# Autodesk Inventor assembly: CNC-FullAssembly
(part 2 of 2)
- Mate:203: SFU1605-BallScrew500mm:2 ↔ BF12-BallScrewStabilizer2:2
- Mate:204: SFU1605-BallScrew500mm:2 ↔ BF12-BallScrewStabilizer2:2
- Flush:119: HGR20R-LinearRail500mm:4 ↔ BF12-BallScrewStabilizer2:2
- Angle:8 (0 deg): 20x40x500mm-Extrusion2:2 ↔ BF12-BallScrewStabilizer2:2
- Mate:205: SFU1605-BallScrew500mm:2 ↔ Nema23-StepperMotor:2
- Angle:9 (0 deg): 20x40x500mm-Extrusion2:2 ↔ Nema23-StepperMotor:2
- Mate:206: Nema23-StepperMotor:2 ↔ MH2025-6.35x10mmCoupler:2
- Mate:207 (2 mm): SFU1605-BallScrew500mm:2 ↔ MH2025-6.35x10mmCoupler:2
- Mate:208 (2 mm): Nema23-StepperMotor:2 ↔ MH2025-6.35x10mmCoupler:2
- Mate:209: SFU1605-BallScrew500mm:2 ↔ BK12-BallScrewStabilizer:2
- Angle:10 (0 deg): HGR20R-LinearRail500mm:4 ↔ BK12-BallScrewStabilizer:2
- Mate:211: 20x40x500mm-Extrusion2:1 ↔ CNC-007-XAxisBallScrewMount:1
- Mate:212: 20x40x500mm-Extrusion2:1 ↔ CNC-007-XAxisBallScrewMount:1
- Mate:213: 20x40x500mm-Extrusion2:1 ↔ CNC-007-XAxisBallScrewMount:1
- Mate:214: CNC-007-XAxisBallScrewMount:1 ↔ 91290A231-M5x15mm:36
- Mate:215: CNC-007-XAxisBallScrewMount:1 ↔ 91290A231-M5x15mm:33
- Mate:216: CNC-007-XAxisBallScrewMount:1 ↔ 91290A231-M5x15mm:34
- Mate:217: CNC-007-XAxisBallScrewMount:1 ↔ 91290A231-M5x15mm:37
- Mate:218: CNC-007-XAxisBallScrewMount:1 ↔ 91290A231-M5x15mm:32
- Mate:219: CNC-007-XAxisBallScrewMount:1 ↔ 91290A231-M5x15mm:31
- Mate:220: CNC-007-XAxisBallScrewMount:1 ↔ 91290A231-M5x15mm:35
- Mate:221: CNC-007-XAxisBallScrewMount:1 ↔ 91290A231-M5x15mm:36
- Flush:120: 91290A231-M5x15mm:33 ↔ 91290A231-M5x15mm:34
- Flush:121: 91290A231-M5x15mm:33 ↔ 91290A231-M5x15mm:37
- Flush:122: 91290A231-M5x15mm:32 ↔ 91290A231-M5x15mm:37
- Flush:123: 91290A231-M5x15mm:31 ↔ 91290A231-M5x15mm:32
- Flush:124: 91290A231-M5x15mm:31 ↔ 91290A231-M5x15mm:35
- Flush:125: 91290A231-M5x15mm:32 ↔ 91290A231-M5x15mm:36
- Mate:222: CNC-007-XAxisBallScrewMount:1 ↔ 91290A231-M5x15mm:38
- Flush:126: 91290A231-M5x15mm:36 ↔ 91290A231-M5x15mm:38
- Mate:223: CNC-007-XAxisBallScrewMount:1 ↔ 91290A231-M5x15mm:39
- Flush:127: 91290A231-M5x15mm:32 ↔ 91290A231-M5x15mm:39
- Mate:224: HGR20R-LinearRail500mm:4 ↔ 91290A231-M5x15mm:40
- Mate:225: HGR20R-LinearRail500mm:4 ↔ 91290A231-M5x15mm:40
- Mate:226: HGR20R-LinearRail500mm:3 ↔ 91290A231-M5x15mm:41
- Flush:128: 91290A231-M5x15mm:41 ↔ 91290A231-M5x15mm:40
- Mate:227: 20x40x500mm-Extrusion2:4 ↔ CNC-008-XAxisNema23Mount:1
- Mate:228: 20x40x500mm-Extrusion2:3 ↔ CNC-008-XAxisNema23Mount:1
- Mate:229: 20x40x500mm-Extrusion2:3 ↔ CNC-008-XAxisNema23Mount:1
- Mate:230: CNC-008-XAxisNema23Mount:1 ↔ 91290A231-M5x15mm:64
- Mate:231: CNC-008-XAxisNema23Mount:1 ↔ 91290A231-M5x15mm:59
- Mate:232: CNC-008-XAxisNema23Mount:1 ↔ 91290A231-M5x15mm:60
- Mate:233: CNC-008-XAxisNema23Mount:1 ↔ 91290A231-M5x15mm:58
- Mate:234: CNC-008-XAxisNema23Mount:1 ↔ 91290A231-M5x15mm:61
- Mate:235: CNC-008-XAxisNema23Mount:1 ↔ 91290A231-M5x15mm:62
- Mate:236: CNC-008-XAxisNema23Mount:1 ↔ 91290A231-M5x15mm:66
- Mate:237: CNC-008-XAxisNema23Mount:1 ↔ 91290A231-M5x15mm:65
- Mate:238: CNC-008-XAxisNema23Mount:1 ↔ 91290A231-M5x15mm:63
- Mate:239: CNC-008-XAxisNema23Mount:1 ↔ 91290A231-M5x15mm:63
- Flush:129: 91290A231-M5x15mm:63 ↔ 91290A231-M5x15mm:65
- Flush:130: 91290A231-M5x15mm:65 ↔ 91290A231-M5x15mm:66
- Flush:131: 91290A231-M5x15mm:62 ↔ 91290A231-M5x15mm:66
- Flush:132: 91290A231-M5x15mm:61 ↔ 91290A231-M5x15mm:62
- Flush:133: 91290A231-M5x15mm:58 ↔ 91290A231-M5x15mm:61
- Flush:134: 91290A231-M5x15mm:58 ↔ 91290A231-M5x15mm:59
- Flush:135: 91290A231-M5x15mm:59 ↔ 91290A231-M5x15mm:64
- Flush:136: 91290A231-M5x15mm:60 ↔ 91290A231-M5x15mm:64
- Mate:240: MH2025-6.35x10mmCoupler:2 ↔ CNC-009-XAxisNema23Spacer:1
- Mate:241: CNC-008-XAxisNema23Mount:1 ↔ CNC-009-XAxisNema23Spacer:1
- Mate:242: CNC-008-XAxisNema23Mount:1 ↔ CNC-009-XAxisNema23Spacer:1
- Mate:243: Nema23-StepperMotor:2 ↔ 91290A198-M5-50mm:2
- Mate:244: Nema23-StepperMotor:2 ↔ 91290A198-M5-50mm:1
- Mate:245: Nema23-StepperMotor:2 ↔ 91290A198-M5-50mm:3
- Mate:246: Nema23-StepperMotor:2 ↔ 91290A198-M5-50mm:4
- Mate:247: Nema23-StepperMotor:2 ↔ 91290A198-M5-50mm:4
- Flush:137: 91290A198-M5-50mm:3 ↔ 91290A198-M5-50mm:4
- Flush:138: 91290A198-M5-50mm:1 ↔ 91290A198-M5-50mm:2
- Flush:139: 91290A198-M5-50mm:2 ↔ 91290A198-M5-50mm:3
- Mate:248: 91290A198-M5-50mm:1 ↔ 90576A104-M5-NylockNut:6
- Mate:249: 91290A198-M5-50mm:4 ↔ 90576A104-M5-NylockNut:8
- Mate:250: 91290A198-M5-50mm:2 ↔ 90576A104-M5-NylockNut:7
- Mate:251: 91290A198-M5-50mm:3 ↔ 90576A104-M5-NylockNut:5
- Mate:252: CNC-008-XAxisNema23Mount:1 ↔ 90576A104-M5-NylockNut:5
- Mate:253: CNC-008-XAxisNema23Mount:1 ↔ 90576A104-M5-NylockNut:8
- Mate:254: CNC-008-XAxisNema23Mount:1 ↔ 90576A104-M5-NylockNut:6
- Mate:255: CNC-008-XAxisNema23Mount:1 ↔ 90576A104-M5-NylockNut:7
- Mate:256: SFU1605-BallScrew500mm:2 ↔ BK12-BallScrewStabilizer:2
- Angle:11 (0 deg): 20x40x500mm-Extrusion2:1 ↔ 3103-0001-0002-GobildaLimitSwitch:1
- Tangent:2: 20x40x500mm-Extrusion2:1 ↔ CNC-010-XAxisLimitSwitchMount:1
- Mate:258: 3103-0001-0002-GobildaLimitSwitch:1 ↔ CNC-010-XAxisLimitSwitchMount:1
- Mate:259: 3103-0001-0002-GobildaLimitSwitch:1 ↔ CNC-010-XAxisLimitSwitchMount:1
- Mate:260: CNC-010-XAxisLimitSwitchMount:1 ↔ 97763A820-M5x10mm-ButtonHead:2
- Mate:261: CNC-010-XAxisLimitSwitchMount:1 ↔ 97763A820-M5x10mm-ButtonHead:2
- Mate:262: CNC-010-XAxisLimitSwitchMount:1 ↔ 97763A820-M5x10mm-ButtonHead:1
- Mate:263: CNC-010-XAxisLimitSwitchMount:1 ↔ 97763A820-M5x10mm-ButtonHead:1
- Mate:264: 40x40x500mm-Extrusion:1 ↔ 91290A231-M5x15mm:22
- Mate:265: CNC-000-StructureGusset1:1 ↔ 90576A104-M5-NylockNut:2
- Mate:269: BF12-BallScrewStabilizer2:1 ↔ CNC-001-StructureGusset2:1
- Flush:142: HGH20-LinearRailCarriage:5 ↔ HGR20R-LinearRail500mm:4
- Tangent:3: 20x20x500mm_Extrusion:3 ↔ CNC-010-XAxisLimitSwitchMount:1
- Flush:143 (-1 mm): 20x40x500mm-Extrusion2:1 ↔ CNC-010-XAxisLimitSwitchMount:1
- Tangent:4: 20x40x500mm-Extrusion2:1 ↔ CNC-011-XAxisHardStop:1
- Tangent:5: 20x20x500mm_Extrusion:3 ↔ CNC-011-XAxisHardStop:1
- Mate:270: 20x40x500mm-Extrusion2:1 ↔ CNC-011-XAxisHardStop:1
- Flush:144 (21.565 mm): 20x20x500mm_Extrusion:3 ↔ CNC-011-XAxisHardStop:1
- Mate:271: CNC-011-XAxisHardStop:1 ↔ 91274A125-M5x8mm:25
- Mate:272: CNC-011-XAxisHardStop:1 ↔ 91274A125-M5x8mm:25
- Mate:273: CNC-011-XAxisHardStop:1 ↔ 91274A125-M5x8mm:26
- Flush:145: 91274A125-M5x8mm:25 ↔ 91274A125-M5x8mm:26
- Mate:274: CNC-011-XAxisHardStop:1 ↔ CNC-011-XAxisHardStop:2
- Mate:275: 91274A125-M5x8mm:26 ↔ CNC-011-XAxisHardStop:2
- Mate:276: 20x40x500mm-Extrusion2:4 ↔ CNC-011-XAxisHardStop:2
- Mate:277: CNC-011-XAxisHardStop:2 ↔ 91274A125-M5x8mm:27
- Mate:278: CNC-011-XAxisHardStop:2 ↔ 91274A125-M5x8mm:28
- Mate:279: CNC-011-XAxisHardStop:2 ↔ 91274A125-M5x8mm:28
- Mate:280: CNC-011-XAxisHardStop:2 ↔ 91274A125-M5x8mm:27
- Mate:281: HGH20-LinearRailCarriage:3 ↔ 91263A832-M5x10mm-Countersink:2
- Mate:282: HGH20-LinearRailCarriage:3 ↔ CNC-005-XAxisMount1:1
- Mate:283: HGH20-LinearRailCarriage:2 ↔ CNC-005-XAxisMount1:1
- Mate:284: HGH20-LinearRailCarriage:1 ↔ 91263A832-M5x10mm-Countersink:6
- Mate:285: HGH20-LinearRailCarriage:4 ↔ CNC-005-XAxisMount1:1
- Mate:286: 40x40x500mm-Extrusion:1 ↔ HGR20R-LinearRail300mm:2
- Flush:146: 40x40x500mm-Extrusion:1 ↔ HGR20R-LinearRail300mm:2
- Mate:287: CNC-000-StructureGusset1:1 ↔ HGR20R-LinearRail300mm:2
- Mate:288: HGR20R-LinearRail300mm:2 ↔ 91290A231-M5x15mm:1
- Mate:289: HGR20R-LinearRail300mm:2 ↔ 91290A231-M5x15mm:1
- Mate:290: 40x40x500mm-Extrusion:2 ↔ HGR20R-LinearRail300mm:1
- Mate:291: CNC-000-StructureGusset1:1 ↔ HGR20R-LinearRail300mm:1
- Flush:147: 40x40x500mm-Extrusion:2 ↔ HGR20R-LinearRail300mm:1
- Mate:292: HGR20R-LinearRail300mm:1 ↔ 91290A231-M5x15mm:83
- Flush:148: 91290A231-M5x15mm:83 ↔ 91290A231-M5x15mm:1
- Mate:293: 40x40x500mm-Extrusion:1 ↔ 20x40x500mm-Extrusion:1
- Mate:294: 40x40x500mm-Extrusion:2 ↔ 20x40x500mm-Extrusion:2
- Mate:295: BK12-BallScrewStabilizer:1 ↔ SFU1605-BallScrew400mm:1
- Mate:296: BK12-BallScrewStabilizer:1 ↔ SFU1605-BallScrew400mm:1
- Mate:297: MH2025-6.35x10mmCoupler:1 ↔ SFU1605-BallScrew400mm:1
- Mate:298: BF12-BallScrewStabilizer2:1 ↔ SFU1605-BallScrew400mm:1
- Mate:299: 40x40x500mm-Extrusion:2 ↔ CNC-001-StructureGusset2:1
- Mate:300: CNC-001-StructureGusset2:1 ↔ CNC-002-ShimStructureGusset2:1
- Mate:301: Nema23-StepperMotor:1 ↔ CNC-004-Nema23Shim:1
- Mate:302: CNC-000-StructureGusset1:1 ↔ 91290A231-M5x15mm:23
- Mate:303: HGH20-LinearRailCarriage:1 ↔ HGR20R-LinearRail300mm:2
- Mate:304: HGH20-LinearRailCarriage:1 ↔ HGR20R-LinearRail300mm:2
- Tangent:7 (78.25 mm): 40x40x500mm-Extrusion:1 ↔ RouterSpindle-65mm:1
- Tangent:8 (171.8503 mm): 20x40x500mm-Extrusion:1 ↔ RouterSpindle-65mm:1
- Mate:305: 3103-0001-0002-GobildaLimitSwitch:1 ↔ 90128A046-#2-.375in:1
- Mate:306: 3103-0001-0002-GobildaLimitSwitch:1 ↔ 90128A046-#2-.375in:2
- Mate:307: CNC-010-XAxisLimitSwitchMount:1 ↔ 90128A046-#2-.375in:2
- Mate:308: CNC-010-XAxisLimitSwitchMount:1 ↔ 90128A046-#2-.375in:1
- Mate:309: 90128A046-#2-.375in:2 ↔ 90480A003-#2-HexNut:1
- Mate:310: 3103-0001-0002-GobildaLimitSwitch:1 ↔ 90480A003-#2-HexNut:1
- Mate:311: 90128A046-#2-.375in:1 ↔ 90480A003-#2-HexNut:2
- Flush:149: 90480A003-#2-HexNut:1 ↔ 90480A003-#2-HexNut:2
- Mate:312: 20x20x500mm_Extrusion:3 ↔ CNC-010-XAxisLimitSwitchMount:1
- Mate:313: HGR20R-LinearRail500mm:4 ↔ 91290A231-M5x15mm:82
- Mate:314: HGR20R-LinearRail500mm:3 ↔ 91290A231-M5x15mm:81
- Angle:12 (0 deg): 40x40x500mm-Extrusion:2 ↔ 3103-0001-0002-GobildaLimitSwitch:2
- Flush:150: HGH20-LinearRailCarriage:3 ↔ 3103-0001-0002-GobildaLimitSwitch:2
- Mate:315 (6.75 mm): 40x40x500mm-Extrusion:2 ↔ 3103-0001-0002-GobildaLimitSwitch:2
- Mate:316: 3103-0001-0002-GobildaLimitSwitch:2 ↔ CNC-012-YAxisLimitSwitchMount:1
- Mate:318: 3103-0001-0002-GobildaLimitSwitch:2 ↔ CNC-012-YAxisLimitSwitchMount:1
- Angle:13 (0 deg): 40x40x500mm-Extrusion:2 ↔ CNC-012-YAxisLimitSwitchMount:1
- Mate:319: CNC-012-YAxisLimitSwitchMount:1 ↔ 90480A003-#2-HexNut:3
- Angle:14 (0 deg): CNC-012-YAxisLimitSwitchMount:1 ↔ 90480A003-#2-HexNut:3
- Mate:320: CNC-012-YAxisLimitSwitchMount:1 ↔ 90480A003-#2-HexNut:3
- Mate:321: 3103-0001-0002-GobildaLimitSwitch:2 ↔ 90480A003-#2-HexNut:4
- Angle:15 (0 deg): CNC-012-YAxisLimitSwitchMount:1 ↔ 90480A003-#2-HexNut:4
- Mate:322: CNC-012-YAxisLimitSwitchMount:1 ↔ 90480A003-#2-HexNut:4
- Mate:323: 3103-0001-0002-GobildaLimitSwitch:2 ↔ 90128A046-#2-.375in:3
- Mate:324: 3103-0001-0002-GobildaLimitSwitch:2 ↔ 90128A046-#2-.375in:4
- Mate:325: 3103-0001-0002-GobildaLimitSwitch:2 ↔ 90128A046-#2-.375in:4
- Flush:151: 90128A046-#2-.375in:3 ↔ 90128A046-#2-.375in:4
- Mate:326: CNC-012-YAxisLimitSwitchMount:1 ↔ 97763A820-M5x10mm-ButtonHead:3
- Mate:327: CNC-012-YAxisLimitSwitchMount:1 ↔ 97763A820-M5x10mm-ButtonHead:4
- Mate:328: CNC-012-YAxisLimitSwitchMount:1 ↔ 97763A820-M5x10mm-ButtonHead:4
- Flush:152: 97763A820-M5x10mm-ButtonHead:3 ↔ 97763A820-M5x10mm-ButtonHead:4
- Mate:329: HGH20-LinearRailCarriage:2 ↔ 20x40x500mm-Extrusion:2
- Flush:153 (30.4587 mm): 40x40x500mm-Extrusion:2 ↔ CNC-012-YAxisLimitSwitchMount:1
